# Autodesk Inventor assembly: Omni Robot
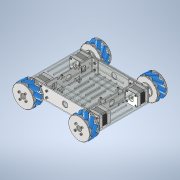
[picture p0: Inventor's stored thumbnail of the model, 180x180]
Saved by Autodesk Inventor 2021 (Build 250183000, 183)
## iProperties
Created: 2022-05-03
Part Number: Omni Robot
Document SubType Name: Assembly
Designer: 21155308
Author: 21155308
## Documents named in this file (12)
- U:\Projeto\Omni Robot.iam
- U:\Projeto\Base.ipt
- U:\Projeto\chapa lateral.ipt
- U:\Projeto\MINEBEA 05701607 stepper motor.ipt
- U:\Projeto\chapa central.ipt
- U:\Projeto\roda direita\Mecanum Wheel Assembly Right-r4.iam
- U:\Projeto\roda esquerda\Mecanum Wheel Assembly Left-r4.iam
- C:\Users\21155308\Documents\Inventor\Content Center Files\R2021\pt-BR\ISO 4762(2)\ISO 4762 - M3 x 5ISO.ipt
- C:\Users\21155308\Documents\Inventor\Content Center Files\R2021\pt-BR\ISO 4762(2)\ISO 4762 - M4 x 10ISO.ipt
- C:\Users\21155308\Documents\Inventor\Content Center Files\R2021\pt-BR\ISO 4032(2)\ISO 4032 - M4 - ISO.ipt
- U:\Projeto\arduino\arduino_MEGA2560.iam
- U:\Projeto\Shield Ramps 1.4.ipt
## Components (56 placed, 11 different names)
1. Base:1 — Coincidente:1, Alinhado:1, Alinhado:3, Coincidente:5, Coincidente:19, Coincidente:21
2. Base:2 — Coincidente:2, Alinhado:2, Coincidente:3, Alinhado:4, Alinhado:5
3. chapa lateral:1 — Coincidente:1, Coincidente:2, Alinhado:1, Alinhado:2, Alinhado:3, Coincidente:3, Coincidente:6, Coincidente:7, Coincidente:8, Coincidente:12, Coincidente:13, Coincidente:14, Coincidente:18, Coincidente:20, Alinhado:7, Coincidente:23, Coincidente:25, Inserir:10, Inserir:11, Inserir:12, Inserir:13, Inserir:14, Inserir:15, Inserir:16, Inserir:17, Inserir:29, Inserir:30, Inserir:31, Inserir:32
4. chapa lateral:2 — Coincidente:5, Alinhado:4, Alinhado:5, Coincidente:9, Coincidente:10, Coincidente:11, Coincidente:15, Coincidente:16, Coincidente:17, Alinhado:6, Coincidente:27, Coincidente:29, Inserir:9, Inserir:18, Inserir:19, Inserir:20, Inserir:21, Inserir:22, Inserir:23, Inserir:24, Inserir:25, Inserir:26, Inserir:27, Inserir:28
5. MINEBEA 05701607 stepper motor:1 — Coincidente:9, Coincidente:10, Coincidente:11, Coincidente:28
6. MINEBEA 05701607 stepper motor:2 — Coincidente:6, Coincidente:7, Coincidente:8, Coincidente:24
7. MINEBEA 05701607 stepper motor:3 — Coincidente:15, Coincidente:16, Coincidente:17, Coincidente:26
8. MINEBEA 05701607 stepper motor:4 — Coincidente:12, Coincidente:13, Coincidente:14, Coincidente:22
9. chapa central:1 — Coincidente:18, Coincidente:19, Alinhado:7, Inserir:1, Inserir:2, Inserir:5, Inserir:8
10. chapa central:2 — Coincidente:20, Coincidente:21, Alinhado:6, Inserir:3, Inserir:4, Inserir:6, Inserir:7
11. Mecanum Wheel Assembly Right-r4:1 [sub-assembly] — Coincidente:22, Coincidente:23
12. Mecanum Wheel Assembly Right-r4:2 [sub-assembly] — Coincidente:28, Coincidente:29
13. Mecanum Wheel Assembly Left-r4:1 [sub-assembly] — Coincidente:24, Coincidente:25
14. Mecanum Wheel Assembly Left-r4:2 [sub-assembly] — Coincidente:26, Coincidente:27
15. ISO 4762 M3 x 5:1 — Inserir:13
16. ISO 4762 M3 x 5:2 — Inserir:12
17. ISO 4762 M3 x 5:3 — Inserir:11
18. ISO 4762 M3 x 5:4 — Inserir:7
19. ISO 4762 M3 x 5:5 — Inserir:8
20. ISO 4762 M3 x 5:6 — Inserir:10
21. ISO 4762 M3 x 5:7 — Inserir:9
22. ISO 4762 M3 x 5:8 — Inserir:14
23. ISO 4762 M3 x 5:9 — Inserir:16
24. ISO 4762 M3 x 5:10 — Inserir:5
25. ISO 4762 M3 x 5:11 — Inserir:1
26. ISO 4762 M3 x 5:12 — Inserir:2
27. ISO 4762 M3 x 5:13 — Inserir:3
28. ISO 4762 M3 x 5:14 — Inserir:4
29. ISO 4762 M3 x 5:15 — Inserir:6
30. ISO 4762 M3 x 5:16 — Inserir:18
31. ISO 4762 M3 x 5:17 — Inserir:17
32. ISO 4762 M3 x 5:18 — Inserir:15
33. ISO 4762 M3 x 5:19 — Inserir:20
34. ISO 4762 M3 x 5:20 — Inserir:19
35. ISO 4762 M3 x 5:21 — Inserir:21
36. ISO 4762 M3 x 5:22 — Inserir:22
37. ISO 4762 M3 x 5:23 — Inserir:23
38. ISO 4762 M3 x 5:24 — Inserir:24
39. ISO 4762 M4 x 10:1 — Inserir:25, Inserir:35
40. ISO 4762 M4 x 10:2 — Inserir:28, Inserir:36
41. ISO 4762 M4 x 10:3 — Inserir:31, Inserir:37
42. ISO 4762 M4 x 10:4 — Inserir:27, Inserir:34
43. ISO 4762 M4 x 10:5 — Inserir:26, Inserir:33
44. ISO 4762 M4 x 10:6 — Inserir:32, Inserir:38
45. ISO 4762 M4 x 10:7 — Inserir:30, Inserir:40
46. ISO 4762 M4 x 10:8 — Inserir:29, Inserir:39
47. ISO 4032 M4:1 — Inserir:35
48. ISO 4032 M4:2 — Inserir:36
49. ISO 4032 M4:3 — Inserir:37
50. ISO 4032 M4:4 — Inserir:34
51. ISO 4032 M4:5 — Inserir:38
52. ISO 4032 M4:6 — Inserir:33
53. ISO 4032 M4:7 — Inserir:40
54. ISO 4032 M4:8 — Inserir:39
55. arduino_MEGA2560:1 [sub-assembly] — Rígida:1
56. Shield Ramps 1.4:1 — Rígida:1
## Relationships (76: Insert 40, Mate 28, Flush 7, WeldJoint 1)
- Coincidente:1 [Mate]: Base:1 ↔ chapa lateral:1
- Coincidente:2 [Mate]: Base:2 ↔ chapa lateral:1
- Alinhado:1 [Flush]: Base:1 ↔ chapa lateral:1
- Alinhado:2 [Flush]: Base:2 ↔ chapa lateral:1
- Alinhado:3 [Flush]: Base:1 ↔ chapa lateral:1
- Coincidente:3 [Mate]: Base:2 ↔ chapa lateral:1
- Coincidente:5 [Mate]: Base:1 ↔ chapa lateral:2
- Alinhado:4 [Flush]: Base:2 ↔ chapa lateral:2
- Alinhado:5 [Flush]: Base:2 ↔ chapa lateral:2
- Coincidente:6 [Mate]: chapa lateral:1 ↔ MINEBEA 05701607 stepper motor:2
- Coincidente:7 [Mate]: chapa lateral:1 ↔ MINEBEA 05701607 stepper motor:2
- Coincidente:8 [Mate]: chapa lateral:1 ↔ MINEBEA 05701607 stepper motor:2
- Coincidente:9 [Mate]: chapa lateral:2 ↔ MINEBEA 05701607 stepper motor:1
- Coincidente:10 [Mate]: chapa lateral:2 ↔ MINEBEA 05701607 stepper motor:1
- Coincidente:11 [Mate]: chapa lateral:2 ↔ MINEBEA 05701607 stepper motor:1
- Coincidente:12 [Mate]: chapa lateral:1 ↔ MINEBEA 05701607 stepper motor:4
- Coincidente:13 [Mate]: chapa lateral:1 ↔ MINEBEA 05701607 stepper motor:4
- Coincidente:14 [Mate]: chapa lateral:1 ↔ MINEBEA 05701607 stepper motor:4
- Coincidente:15 [Mate]: chapa lateral:2 ↔ MINEBEA 05701607 stepper motor:3
- Coincidente:16 [Mate]: chapa lateral:2 ↔ MINEBEA 05701607 stepper motor:3
- Coincidente:17 [Mate]: chapa lateral:2 ↔ MINEBEA 05701607 stepper motor:3
- Coincidente:18 [Mate]: chapa lateral:1 ↔ chapa central:1
- Coincidente:19 [Mate]: Base:1 ↔ chapa central:1
- Coincidente:20 [Mate]: chapa lateral:1 ↔ chapa central:2
- Coincidente:21 [Mate]: Base:1 ↔ chapa central:2
- Alinhado:6 [Flush] (42 mm): chapa lateral:2 ↔ chapa central:2
- Alinhado:7 [Flush] (42 mm): chapa lateral:1 ↔ chapa central:1
- Coincidente:22 [Mate]: MINEBEA 05701607 stepper motor:4 ↔ Mecanum Wheel Assembly Right-r4:1
- Coincidente:23 [Mate] (10 mm): chapa lateral:1 ↔ Mecanum Wheel Assembly Right-r4:1
- Coincidente:24 [Mate]: MINEBEA 05701607 stepper motor:2 ↔ Mecanum Wheel Assembly Left-r4:1
- Coincidente:25 [Mate] (10 mm): chapa lateral:1 ↔ Mecanum Wheel Assembly Left-r4:1
- Coincidente:26 [Mate]: MINEBEA 05701607 stepper motor:3 ↔ Mecanum Wheel Assembly Left-r4:2
- Coincidente:27 [Mate] (10 mm): chapa lateral:2 ↔ Mecanum Wheel Assembly Left-r4:2
- Coincidente:28 [Mate]: MINEBEA 05701607 stepper motor:1 ↔ Mecanum Wheel Assembly Right-r4:2
- Coincidente:29 [Mate] (10 mm): chapa lateral:2 ↔ Mecanum Wheel Assembly Right-r4:2
- Inserir:1 (1.3 mm): chapa central:1 ↔ ISO 4762 M3 x 5:11
- Inserir:2 (1.3 mm): chapa central:1 ↔ ISO 4762 M3 x 5:12
- Inserir:3 (1.3 mm): chapa central:2 ↔ ISO 4762 M3 x 5:13
- Inserir:4 (1.3 mm): chapa central:2 ↔ ISO 4762 M3 x 5:14
- Inserir:5 (1.3 mm): chapa central:1 ↔ ISO 4762 M3 x 5:10
- Inserir:6 (1.3 mm): chapa central:2 ↔ ISO 4762 M3 x 5:15
- Inserir:7 (1.3 mm): chapa central:2 ↔ ISO 4762 M3 x 5:4
- Inserir:8 (1.3 mm): chapa central:1 ↔ ISO 4762 M3 x 5:5
- Inserir:9 (-4.6 mm): chapa lateral:2 ↔ ISO 4762 M3 x 5:7
- Inserir:10 (-4.6 mm): chapa lateral:1 ↔ ISO 4762 M3 x 5:6
- Inserir:11 (-4.6 mm): chapa lateral:1 ↔ ISO 4762 M3 x 5:3
- Inserir:12 (-4.6 mm): chapa lateral:1 ↔ ISO 4762 M3 x 5:2
- Inserir:13 (-4.6 mm): chapa lateral:1 ↔ ISO 4762 M3 x 5:1
- Inserir:14 (-4.6 mm): chapa lateral:1 ↔ ISO 4762 M3 x 5:8
- Inserir:15 (-4.6 mm): chapa lateral:1 ↔ ISO 4762 M3 x 5:18
- Inserir:16 (-4.6 mm): chapa lateral:1 ↔ ISO 4762 M3 x 5:9
- Inserir:17 (-4.6 mm): chapa lateral:1 ↔ ISO 4762 M3 x 5:17
- Inserir:18 (-4.6 mm): chapa lateral:2 ↔ ISO 4762 M3 x 5:16
- Inserir:19 (-4.6 mm): chapa lateral:2 ↔ ISO 4762 M3 x 5:20
- Inserir:20 (-4.6 mm): chapa lateral:2 ↔ ISO 4762 M3 x 5:19
- Inserir:21 (-4.6 mm): chapa lateral:2 ↔ ISO 4762 M3 x 5:21
- Inserir:22 (-4.6 mm): chapa lateral:2 ↔ ISO 4762 M3 x 5:22
- Inserir:23 (-4.6 mm): chapa lateral:2 ↔ ISO 4762 M3 x 5:23
- Inserir:24 (-4.6 mm): chapa lateral:2 ↔ ISO 4762 M3 x 5:24
- Inserir:25 (-6.5 mm): chapa lateral:2 ↔ ISO 4762 M4 x 10:1
- Inserir:26 (-6.5 mm): chapa lateral:2 ↔ ISO 4762 M4 x 10:5
- Inserir:27 (-6.5 mm): chapa lateral:2 ↔ ISO 4762 M4 x 10:4
- Inserir:28 (-6.5 mm): chapa lateral:2 ↔ ISO 4762 M4 x 10:2
- Inserir:29 (-6.5 mm): chapa lateral:1 ↔ ISO 4762 M4 x 10:8
- Inserir:30 (-6.5 mm): chapa lateral:1 ↔ ISO 4762 M4 x 10:7
- Inserir:31 (-6.5 mm): chapa lateral:1 ↔ ISO 4762 M4 x 10:3
- Inserir:32 (-6.5 mm): chapa lateral:1 ↔ ISO 4762 M4 x 10:6
- Inserir:33: ISO 4762 M4 x 10:5 ↔ ISO 4032 M4:6
- Inserir:34: ISO 4762 M4 x 10:4 ↔ ISO 4032 M4:4
- Inserir:35: ISO 4762 M4 x 10:1 ↔ ISO 4032 M4:1
- Inserir:36: ISO 4762 M4 x 10:2 ↔ ISO 4032 M4:2
- Inserir:37: ISO 4762 M4 x 10:3 ↔ ISO 4032 M4:3
- Inserir:38: ISO 4762 M4 x 10:6 ↔ ISO 4032 M4:5
- Inserir:39: ISO 4762 M4 x 10:8 ↔ ISO 4032 M4:8
- Inserir:40: ISO 4762 M4 x 10:7 ↔ ISO 4032 M4:7
- Rígida:1 [WeldJoint] (-0.5 mm): arduino_MEGA2560:1 ↔ Shield Ramps 1.4:1
